# Autodesk Inventor assembly: Beginning_assembly
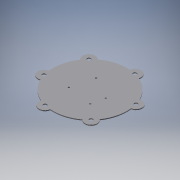
[picture p0: Inventor's stored thumbnail of the model, 180x180]
Saved by Autodesk Inventor 2016 (Build 200138000, 138)
## iProperties
Created: 2015-10-08
Part Number: Beginning_assembly
Document SubType Name: Assembly
Designer: powasar16
Author: powasar16
## Documents named in this file (4)
- C:\Users\powasar16\Documents\GitHub\SpyderRobot\Inventor\Created Parts\Beginning_assembly.iam
- C:\Users\powasar16\Documents\GitHub\SpyderRobot\Inventor\Created Parts\Arduino.ipt
- C:\Users\powasar16\Documents\GitHub\SpyderRobot\Inventor\Created Parts\Base_bottom.ipt
- C:\Users\powasar16\Documents\GitHub\SpyderRobot\Inventor\Imported Parts\Motherboard Standoff 12mm M3x0.5.ipt
## Components (6 placed, 3 different names)
1. Arduino:1 — Mate:1
2. Base_bottom:1 — Mate:1
3. Motherboard Standoff 12mm M3x0.5:1
4. Motherboard Standoff 12mm M3x0.5:2
5. Motherboard Standoff 12mm M3x0.5:3
6. Motherboard Standoff 12mm M3x0.5:4
## Relationships (1: Mate 1)
- Mate:1: Arduino:1 ↔ Base_bottom:1
